# Autodesk Inventor assembly: structure_channel
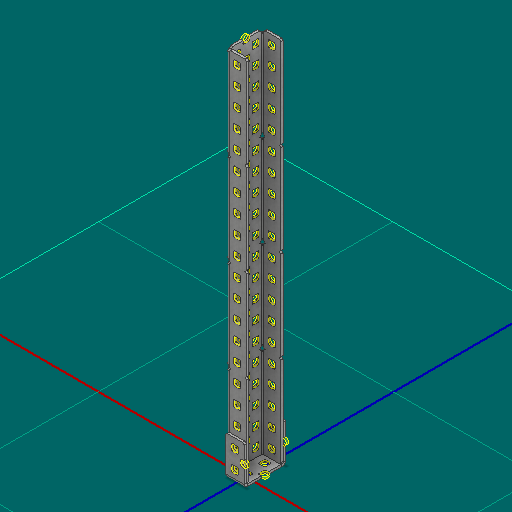
[picture p0: Inventor's stored thumbnail of the model, 512x512]
Saved by Autodesk Inventor 2025 (Build 290162000, 162)
## iProperties
Created: 2024-08-23
Part Number: structure_channel
Document SubType Name: Assembly
Designer: averey
Author: averey
## Documents named in this file (3)
- C:\Users\avere\vex_robotics_high_stakes\hardware\cad\bots\ENIGMA\tower\structure_channel.iam
- C:\Users\avere\vex_robotics_high_stakes\hardware\cad\VEX-CAD-Inventor\Structure\C Channel\Aluminum 2x2x2\Alu C 2x2x2x1.ipt
- C:\Users\avere\vex_robotics_high_stakes\hardware\cad\VEX-CAD-Inventor\Structure\C Channel\Aluminum 1x2x1\Alu C 1x2x1x20.ipt
## Components (2 placed, 2 different names)
1. Alu C 2x2x2x1:1 — Angle:1, Insert:1, Mate:1
2. Alu C 1x2x1x20:1 — Insert:1, Mate:1
## Relationships (3: Angle 1, Insert 1, Mate 1)
- Angle:1 (0 deg): Alu C 2x2x2x1:1
- Insert:1: Alu C 2x2x2x1:1 ↔ Alu C 1x2x1x20:1
- Mate:1: Alu C 2x2x2x1:1 ↔ Alu C 1x2x1x20:1
